# Autodesk Inventor assembly: Ensamblaje1
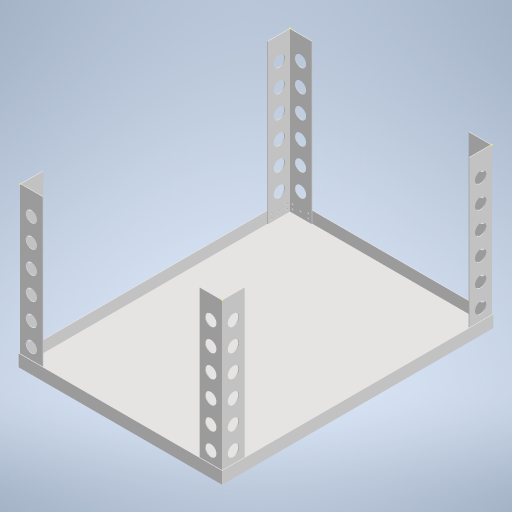
[picture p0: Inventor's stored thumbnail of the model, 512x512]
Saved by Autodesk Inventor 2024 (Build 280153000, 153)
## iProperties
Created: 2023-10-22
Part Number: Ensamblaje1
Document SubType Name: Assembly
Designer: jhonc
Author: jhonc
## Documents named in this file (3)
- C:\Users\jhonc\OneDrive\Escritorio\3 apm\Ensamblaje1.iam
- C:\Users\jhonc\OneDrive\Escritorio\3 apm\tapa mesa.ipt
- C:\Users\jhonc\OneDrive\Escritorio\3 apm\patas.ipt
## Components (5 placed, 2 different names)
1. tapa mesa:1 — Coincidencia:1, Coincidencia:2, Coincidencia:3, Coincidencia:4, Coincidencia:5, Coincidencia:6, Coincidencia:7, Coincidencia:8, Coincidencia:10, Coincidencia:11, Coincidencia:12, Coincidencia:13
2. patas:1 — Coincidencia:2, Coincidencia:5, Coincidencia:6
3. patas:2 — Coincidencia:1, Coincidencia:7, Coincidencia:8
4. patas:3 — Coincidencia:4, Coincidencia:10, Coincidencia:11
5. patas:4 — Coincidencia:3, Coincidencia:12, Coincidencia:13
## Relationships (12: Mate 12)
- Coincidencia:1 [Mate]: tapa mesa:1 ↔ patas:2
- Coincidencia:2 [Mate]: tapa mesa:1 ↔ patas:1
- Coincidencia:3 [Mate]: tapa mesa:1 ↔ patas:4
- Coincidencia:4 [Mate]: tapa mesa:1 ↔ patas:3
- Coincidencia:5 [Mate]: tapa mesa:1 ↔ patas:1
- Coincidencia:6 [Mate]: tapa mesa:1 ↔ patas:1
- Coincidencia:7 [Mate]: tapa mesa:1 ↔ patas:2
- Coincidencia:8 [Mate]: tapa mesa:1 ↔ patas:2
- Coincidencia:10 [Mate]: tapa mesa:1 ↔ patas:3
- Coincidencia:11 [Mate]: tapa mesa:1 ↔ patas:3
- Coincidencia:12 [Mate]: tapa mesa:1 ↔ patas:4
- Coincidencia:13 [Mate]: tapa mesa:1 ↔ patas:4
